# Autodesk Inventor assembly: Estructura
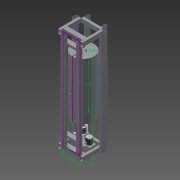
[picture p0: Inventor's stored thumbnail of the model, 180x180]
Saved by Autodesk Inventor 2019 (Build 230136000, 136)
## iProperties
Created: 2019-11-05
Part Number: Estructura
Document SubType Name: Assembly
Designer: Charlie
Author: Charlie
## Documents named in this file (13)
- D:\Drives\OneDrive\Carlos_2\02 TRABAJOS\MULTIPLO\Conveyor\Torno_rodillos\Estructura.iam
- D:\Drives\OneDrive\Carlos_2\02 TRABAJOS\MULTIPLO\Conveyor\Torno_rodillos\sketch_estructura-1-01.ipt
- D:\Drives\OneDrive\Carlos_2\02 TRABAJOS\MULTIPLO\Conveyor\Perfil 30x50.ipt
- Perfil 30x50.ipt
- D:\Drives\OneDrive\Carlos_2\02 TRABAJOS\MULTIPLO\Conveyor\Torno_rodillos\Perfil 30x501.ipt
- D:\Drives\OneDrive\Carlos_2\02 TRABAJOS\MULTIPLO\Conveyor\Torno_rodillos\Perfil 30x502.ipt
- D:\Drives\OneDrive\Carlos_2\02 TRABAJOS\MULTIPLO\Conveyor\Torno_rodillos\ASM_guia_eliptica.iam
- D:\Drives\OneDrive\Carlos_2\02 TRABAJOS\MULTIPLO\Conveyor\Torno_rodillos\chinese-cnc-rotation-axis-module-with-80mm-chuck-1.snapshot.5\globe bot\A_axis_right.iam
- D:\Drives\OneDrive\Carlos_2\02 TRABAJOS\MULTIPLO\Conveyor\Torno_rodillos\Guia eliptica.ipt
- D:\Drives\OneDrive\Carlos_2\02 TRABAJOS\MULTIPLO\Conveyor\Torno_rodillos\Perfil 30x505.ipt
- D:\Drives\OneDrive\Carlos_2\02 TRABAJOS\MULTIPLO\Conveyor\Torno_rodillos\Perfil 30x506.ipt
- D:\Drives\OneDrive\Carlos_2\02 TRABAJOS\MULTIPLO\Conveyor\Torno_rodillos\Perfil 30x507.ipt
- D:\Drives\OneDrive\Carlos_2\02 TRABAJOS\MULTIPLO\Conveyor\Torno_rodillos\soporte inferior ridgid -2.ipt
## Components (22 placed, 10 different names)
1. sketch_estructura-1-01:1 — Mate:19
2. Perfil 30x501:1 — Flush:3, Flush:5, Mate:26, Flush:30, Flush:32, Flush:36
3. Perfil 30x501:2 — Flush:4, Flush:13, Mate:24, Flush:29
4. Perfil 30x502:3 — Flush:1, Flush:2, Flush:3, Flush:4, Flush:23, Mate:19, Mate:24, Flush:29, Mate:25, Mate:26, Flush:30, Mate:27, Flush:37, Mate:33, Flush:41, Flush:44
5. Perfil 30x502:4 — Flush:1, Flush:2, Flush:5, Mate:4, Flush:38, Mate:32, Flush:39, Mate:34, Flush:42, Flush:43
6. Perfil 30x501:5 — Mate:11, Mate:12, Flush:19, Flush:20, Flush:21, Flush:36
7. Perfil 30x501:6 — Flush:18, Mate:16, Flush:24
8. Perfil 30x502:7 — Mate:11, Flush:17, Mate:13, Flush:20
9. Perfil 30x502:8 — Mate:12, Flush:17, Flush:18, Mate:14, Flush:19, Mate:16, Flush:21, Flush:23, Flush:24, Angle:2, Mate:31
10. Perfil 30x501:9 — Flush:13, Mate:25, Mate:29, Mate:38
11. Perfil 30x501:10 — Mate:27, Flush:32
12. ASM_guia_eliptica:1 [sub-assembly] — Mate:13
13. ASM_guia_eliptica:2 [sub-assembly] — Mate:14
14. A_axis_right:1 [sub-assembly] — Mate:17, Mate:29, Mate:30, Mate:38
15. Guia eliptica:1 — Mate:17, Angle:2, Mate:30, Mate:37
16. Perfil 30x507:11 — Mate:31, Flush:37, Flush:40, Mate:35
17. Perfil 30x506:12 — Flush:38, Mate:32, Flush:39, Flush:40, Mate:36
18. Perfil 30x505:13 — Mate:33, Flush:41, Flush:44
19. Perfil 30x505:14 — Mate:34, Flush:42, Flush:43
20. Perfil 30x502:15 — Mate:35
21. Perfil 30x502:16 — Mate:36
22. soporte inferior ridgid -2:1 — Mate:37
## Relationships (48: Flush 25, Mate 22, Angle 1)
- Flush:1: Perfil 30x502:3 ↔ Perfil 30x502:4
- Flush:2: Perfil 30x502:3 ↔ Perfil 30x502:4
- Flush:3: Perfil 30x501:1 ↔ Perfil 30x502:3
- Flush:4: Perfil 30x501:2 ↔ Perfil 30x502:3
- Flush:5: Perfil 30x501:1 ↔ Perfil 30x502:4
- Mate:4: Perfil 30x502:4
- Flush:13: Perfil 30x501:2 ↔ Perfil 30x501:9
- Mate:11: Perfil 30x501:5 ↔ Perfil 30x502:7
- Mate:12: Perfil 30x501:5 ↔ Perfil 30x502:8
- Flush:17: Perfil 30x502:7 ↔ Perfil 30x502:8
- Flush:18: Perfil 30x501:6 ↔ Perfil 30x502:8
- Mate:13: Perfil 30x502:7 ↔ ASM_guia_eliptica:1
- Mate:14: Perfil 30x502:8 ↔ ASM_guia_eliptica:2
- Flush:19: Perfil 30x501:5 ↔ Perfil 30x502:8
- Flush:20: Perfil 30x501:5 ↔ Perfil 30x502:7
- Mate:16: Perfil 30x501:6 ↔ Perfil 30x502:8
- Flush:21: Perfil 30x501:5 ↔ Perfil 30x502:8
- Flush:23: Perfil 30x502:3 ↔ Perfil 30x502:8
- Flush:24: Perfil 30x501:6 ↔ Perfil 30x502:8
- Mate:17: A_axis_right:1 ↔ Guia eliptica:1
- Mate:19: sketch_estructura-1-01:1 ↔ Perfil 30x502:3
- Angle:2 (0 deg): Perfil 30x502:8 ↔ Guia eliptica:1
- Mate:24: Perfil 30x501:2 ↔ Perfil 30x502:3
- Flush:29: Perfil 30x501:2 ↔ Perfil 30x502:3
- Mate:25: Perfil 30x502:3 ↔ Perfil 30x501:9
- Mate:26: Perfil 30x501:1 ↔ Perfil 30x502:3
- Flush:30: Perfil 30x501:1 ↔ Perfil 30x502:3
- Mate:27: Perfil 30x502:3 ↔ Perfil 30x501:10
- Flush:32: Perfil 30x501:1 ↔ Perfil 30x501:10
- Mate:29: Perfil 30x501:9 ↔ A_axis_right:1
- Mate:30: A_axis_right:1 ↔ Guia eliptica:1
- Flush:36: Perfil 30x501:1 ↔ Perfil 30x501:5
- Mate:31: Perfil 30x502:8 ↔ Perfil 30x507:11
- Flush:37: Perfil 30x502:3 ↔ Perfil 30x507:11
- Flush:38: Perfil 30x502:4 ↔ Perfil 30x506:12
- Mate:32: Perfil 30x502:4 ↔ Perfil 30x506:12
- Flush:39: Perfil 30x502:4 ↔ Perfil 30x506:12
- Flush:40: Perfil 30x507:11 ↔ Perfil 30x506:12
- Mate:33: Perfil 30x502:3 ↔ Perfil 30x505:13
- Flush:41: Perfil 30x502:3 ↔ Perfil 30x505:13
- Mate:34: Perfil 30x502:4 ↔ Perfil 30x505:14
- Flush:42: Perfil 30x502:4 ↔ Perfil 30x505:14
- Flush:43: Perfil 30x502:4 ↔ Perfil 30x505:14
- Flush:44: Perfil 30x502:3 ↔ Perfil 30x505:13
- Mate:35: Perfil 30x507:11 ↔ Perfil 30x502:15
- Mate:36: Perfil 30x506:12 ↔ Perfil 30x502:16
- Mate:37: Guia eliptica:1 ↔ soporte inferior ridgid -2:1
- Mate:38 (4 mm): Perfil 30x501:9 ↔ A_axis_right:1
